# Autodesk Inventor assembly: KBHandle
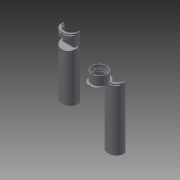
[picture p0: Inventor's stored thumbnail of the model, 180x180]
Saved by Autodesk Inventor 2014 SP2 (Build 180246200, 246)
## iProperties
Created: 2014-08-19
Part Number: KBHandle
Document SubType Name: Assembly
Designer: jkao
Author: jkao
## Documents named in this file (4)
- C:\Users\jkao\Dropbox\inventor\KBHandle\KBHandle.iam
- C:\Users\jkao\Dropbox\inventor\KBHandle\DiffuserCoupler.ipt
- C:\Users\jkao\Dropbox\inventor\KBHandle\Handle-Bottom.ipt
- C:\Users\jkao\Dropbox\inventor\KBHandle\Handle-Top.ipt
## Components (3 placed, 3 different names)
1. DiffuserCoupler:1
2. Handle-Bottom:1
3. Handle-Top:1 — Flush:1
## Relationships (1: Flush 1)
- Flush:1: Handle-Top:1
